# Autodesk Inventor assembly: Assembly1
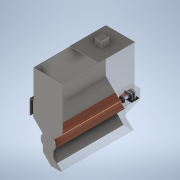
[picture p0: Inventor's stored thumbnail of the model, 180x180]
Saved by Autodesk Inventor 2020 (Build 240168000, 168)
## iProperties
Created: 2020-04-30
Part Number: Assembly1
Document SubType Name: Assembly
Designer: LENOVO
Author: LENOVO
## Documents named in this file (13)
- C:\Users\LENOVO\Desktop\Graduation Project\Fish Farming Unit\foodstorage\Assembly1.iam
- C:\Users\LENOVO\Desktop\Graduation Project\Fish Farming Unit\foodstorage\back.ipt
- C:\Users\LENOVO\Desktop\Graduation Project\Fish Farming Unit\foodstorage\leftside0.ipt
- C:\Users\LENOVO\Desktop\Graduation Project\Fish Farming Unit\foodstorage\rightside0.ipt
- C:\Users\LENOVO\Desktop\Graduation Project\Fish Farming Unit\foodstorage\front.ipt
- C:\Users\LENOVO\Desktop\Graduation Project\Fish Farming Unit\foodstorage\propeller.ipt
- C:\Users\LENOVO\Desktop\Graduation Project\Fish Farming Unit\foodstorage\shaft.ipt
- C:\Users\LENOVO\Desktop\Graduation Project\Fish Farming Unit\foodstorage\tankholder.ipt
- C:\Users\LENOVO\Desktop\Graduation Project\Fish Farming Unit\Feeding Mechanism\Stepper_with_Bracket.iam
- C:\Users\LENOVO\Desktop\Graduation Project\Fish Farming Unit\Feeding Mechanism\Encoder_Disk.ipt
- C:\Users\LENOVO\Desktop\Graduation Project\Fish Farming Unit\Feeding Mechanism\photointerrupter.ipt
- C:\Users\LENOVO\Desktop\Graduation Project\Fish Farming Unit\foodstorage\top_sensor.ipt
- C:\Users\LENOVO\Desktop\Graduation Project\Fish Farming Unit\Feeding Mechanism\HC-SR04_ultrasonic.iam
## Components (12 placed, 12 different names)
1. back:2 — Mate:1, Mate:2, Mate:3, Mate:4, Mate:5, Mate:6, Insert:2, Mate:12
2. leftside0:1 — Mate:1, Mate:2, Mate:3, Mate:7, Mate:8, Mate:9, Mate:13
3. rightside0:1 — Mate:4, Mate:5, Mate:6, Insert:5, Mate:15
4. front:1 — Mate:7, Mate:8, Mate:9, Mate:14
5. propeller:1 — Insert:1, Mate:10, Mate:11, Insert:2
6. shaft:1 — Insert:1, Mate:10, Mate:11, Insert:3, Insert:4
7. tankholder:1 — Mate:12, Mate:13
8. top_sensor:1 — Mate:14, Mate:15, Insert:6
9. Stepper_with_Bracket:1 [sub-assembly] — Insert:3
10. Encoder_Disk:1 — Insert:4
11. photointerrupter:1 — Insert:5
12. HC-SR04_ultrasonic:2 [sub-assembly] — Insert:6
## Relationships (21: Mate 15, Insert 6)
- Mate:1: back:2 ↔ leftside0:1
- Mate:2: back:2 ↔ leftside0:1
- Mate:3: back:2 ↔ leftside0:1
- Mate:4: back:2 ↔ rightside0:1
- Mate:5: back:2 ↔ rightside0:1
- Mate:6: back:2 ↔ rightside0:1
- Mate:7: leftside0:1 ↔ front:1
- Mate:8: leftside0:1 ↔ front:1
- Mate:9: leftside0:1 ↔ front:1
- Insert:1 (-514 mm): propeller:1 ↔ shaft:1
- Mate:10: propeller:1 ↔ shaft:1
- Mate:11: propeller:1 ↔ shaft:1
- Insert:2 (-494 mm): back:2 ↔ propeller:1
- Mate:12: back:2 ↔ tankholder:1
- Mate:13: leftside0:1 ↔ tankholder:1
- Insert:3 (-10 mm): shaft:1 ↔ Stepper_with_Bracket:1
- Insert:4 (14.2 mm): shaft:1 ↔ Encoder_Disk:1
- Insert:5: rightside0:1 ↔ photointerrupter:1
- Mate:14: front:1 ↔ top_sensor:1
- Mate:15: rightside0:1 ↔ top_sensor:1
- Insert:6 (-10 mm): top_sensor:1 ↔ HC-SR04_ultrasonic:2
